# Autodesk Inventor assembly: 75mm Stroke Pneumatic Cylinder.f3d
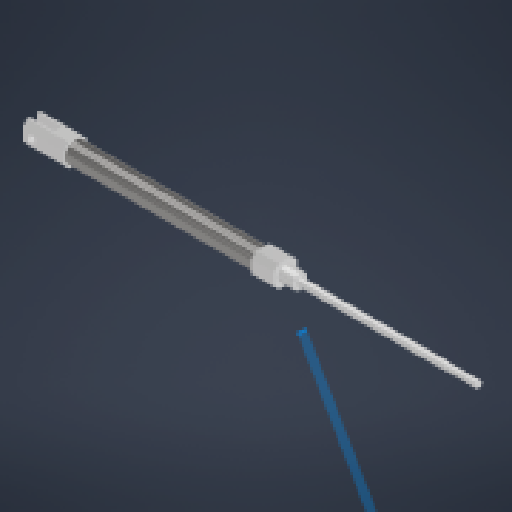
[picture p0: Inventor's stored thumbnail of the model, 512x512]
Saved by Autodesk Inventor 2026.1 (Build 301233000, 233)
## iProperties
Created: 2024-01-30
Part Number: 75mm Stroke Pneumatic Cylinder.f3d
Document SubType Name: Assembly
Designer: AdminForWorker
Title: 75mm Stroke Pneumatic Cylinder.f3d v1
Author: AdminForWorker
## Documents named in this file (3)
- C:\Users\roejo\OneDrive\Documents\7700RKalahariCAD\Library\VEX-CAD-Inventor-1.4.2\Motion\Pneumatics\New - V5 Pneumatics\75mm Stroke Pneumatic Cylinder.iam
- C:\Users\roejo\OneDrive\Documents\7700RKalahariCAD\Library\VEX-CAD-Inventor-1.4.2\Motion\Pneumatics\Reference Parts\Pistons\75mm Piston Body.ipt
- C:\Users\roejo\OneDrive\Documents\7700RKalahariCAD\Library\VEX-CAD-Inventor-1.4.2\Motion\Pneumatics\Reference Parts\Pistons\75mm Piston Rod.ipt
## Components (2 placed, 2 different names)
1. Component1:1 — Cylindrical:1
2. Component2:1 — Cylindrical:1
## Relationships (1: CylindricalJoint 1)
- Cylindrical:1: Component1:1 ↔ Component2:1
